# Autodesk Inventor assembly: Assembly1
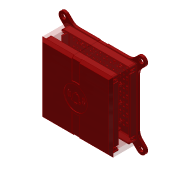
[picture p0: Inventor's stored thumbnail of the model, 180x180]
Saved by Autodesk Inventor 2018 (Build 220112000, 112)
## iProperties
Created: 2017-12-16
Part Number: Assembly1
Document SubType Name: Assembly
Designer: Gebruiker
Author: Gebruiker
## Documents named in this file (4)
- C:\Users\Gebruiker\Documents\school\3dejaar\ap_valley\3D_design\Assembly1.iam
- C:\Users\Gebruiker\Documents\school\3dejaar\ap_valley\3D_design\AP-01.ipt
- C:\Users\Gebruiker\Documents\school\3dejaar\ap_valley\3D_design\AP-02.ipt
- C:\Users\Gebruiker\Documents\school\3dejaar\ap_valley\3D_design\AP-03.ipt
## Components (3 placed, 3 different names)
1. AP-01:1 — Mate:1, Flush:3, Flush:6
2. AP-02:1 — Mate:1, Flush:3, Flush:4, Flush:5, Flush:6, Mate:2
3. AP-03:1 — Flush:4, Flush:5, Mate:2
## Relationships (6: Flush 4, Mate 2)
- Mate:1: AP-01:1 ↔ AP-02:1
- Flush:3: AP-01:1 ↔ AP-02:1
- Flush:4: AP-02:1 ↔ AP-03:1
- Flush:5: AP-02:1 ↔ AP-03:1
- Flush:6: AP-01:1 ↔ AP-02:1
- Mate:2: AP-02:1 ↔ AP-03:1
